# Autodesk Inventor assembly: 002 - Крепление СБ
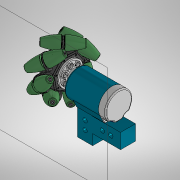
[picture p0: Inventor's stored thumbnail of the model, 180x180]
Saved by Autodesk Inventor 2022 (Build 260153000, 153)
## iProperties
RuleStatus: InUse
Created: 2022-01-16
Part Number: 002 - Крепление СБ
Document SubType Name: Assembly
Designer: Петров Иван
Author: Петров Иван
## Documents named in this file (7)
- E:\IVAN\Ivan_desktop\Kvantorium\Projects\YouBotRobot\design\000.001.002 - Крепление СБ.iam
- E:\IVAN\Ivan_desktop\Kvantorium\Projects\YouBotRobot\design\standart_components\dc_gear_motor_12V_500rpm.ipt
- E:\IVAN\Ivan_desktop\Kvantorium\Projects\YouBotRobot\design\000.001.002.001 - Крепление.ipt
- E:\IVAN\Ivan_desktop\Kvantorium\Projects\YouBotRobot\design\000.001.002.002- Крышка мотора.ipt
- E:\IVAN\Ivan_desktop\Kvantorium\Projects\YouBotRobot\design\standart_components\VEX Meccanum wheel\Rueda 1.ipt
- E:\IVAN\Ivan_desktop\Kvantorium\Projects\YouBotRobot\design\standart_components\vex_mechanum_adapter.ipt
- E:\IVAN\Ivan_desktop\Kvantorium\Projects\YouBotRobot\design\standart_components\vex_mechanum_adapter (1) зеркальный.ipt
## Components (6 placed, 6 different names)
1. dc_gear_motor_12V_500rpm:1 — Совмещение:1, Совмещение:2, Совмещение:3, Совмещение:11, Совмещение:12
2. 000.001.002.001 - Крепление:1 — Совмещение:1, Совмещение:2, Совмещение:3, Совмещение:5, Совмещение:6, Совмещение:7
3. 000.001.002.002- Крышка мотора:1 — Совмещение:5, Совмещение:6, Совмещение:7
4. Rueda 1:1 — Совмещение:8, Совмещение:9, Совмещение:10, Совмещение:13, Совмещение:15
5. vex_mechanum_adapter:1 — Совмещение:8, Совмещение:9, Совмещение:10, Совмещение:11, Совмещение:12, Совмещение:14
6. vex_mechanum_adapter (1) зеркальный:1 — Совмещение:13, Совмещение:14, Совмещение:15
## Relationships (14: Mate 14)
- Совмещение:1 [Mate]: dc_gear_motor_12V_500rpm:1 ↔ 000.001.002.001 - Крепление:1
- Совмещение:2 [Mate]: dc_gear_motor_12V_500rpm:1 ↔ 000.001.002.001 - Крепление:1
- Совмещение:3 [Mate]: dc_gear_motor_12V_500rpm:1 ↔ 000.001.002.001 - Крепление:1
- Совмещение:5 [Mate]: 000.001.002.001 - Крепление:1 ↔ 000.001.002.002- Крышка мотора:1
- Совмещение:6 [Mate]: 000.001.002.001 - Крепление:1 ↔ 000.001.002.002- Крышка мотора:1
- Совмещение:7 [Mate]: 000.001.002.001 - Крепление:1 ↔ 000.001.002.002- Крышка мотора:1
- Совмещение:8 [Mate]: Rueda 1:1 ↔ vex_mechanum_adapter:1
- Совмещение:9 [Mate]: Rueda 1:1 ↔ vex_mechanum_adapter:1
- Совмещение:10 [Mate]: Rueda 1:1 ↔ vex_mechanum_adapter:1
- Совмещение:11 [Mate]: dc_gear_motor_12V_500rpm:1 ↔ vex_mechanum_adapter:1
- Совмещение:12 [Mate]: dc_gear_motor_12V_500rpm:1 ↔ vex_mechanum_adapter:1
- Совмещение:13 [Mate]: Rueda 1:1 ↔ vex_mechanum_adapter (1) зеркальный:1
- Совмещение:14 [Mate]: vex_mechanum_adapter:1 ↔ vex_mechanum_adapter (1) зеркальный:1
- Совмещение:15 [Mate]: Rueda 1:1 ↔ vex_mechanum_adapter (1) зеркальный:1
